# Autodesk Inventor assembly: Channel
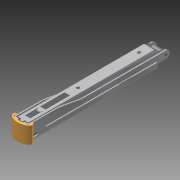
[picture p0: Inventor's stored thumbnail of the model, 180x180]
Saved by Autodesk Inventor 2011 (Build 150239000, 239)
## iProperties
Shininess: 64.0
Length Units: 11272
Angle Units: 11279
Time Units: 11290
Mass Units: 11286
Length Display Precision: 3
Angle Display Precision: 2
Compacted: True
Part Number: Channel
Document SubType Name: Assembly
Created: 2002-09-26
Designer: Autodesk, Inc.
Project: Inventor Samples
Mass: 81.6929 g
Surface Area: 254.71 cm^2
Volume: 11.1757 cm^3
Density: 7.30984 g/cm^3
Density: 0.0
Volumn: 0.0
Area: 0.0
PropertySet Name: Model Information
Control State: 0
Master: False
Checked Out: False
Author: Autodesk, Inc.
Revision Number: A
## Documents named in this file (7)
- C:\Users\Public\Documents\Autodesk\Inventor 2011\Samples\Models\Assemblies\Stapler\Components\Channel.iam
- C:\Users\Public\Documents\Autodesk\Inventor 2011\Samples\Models\Assemblies\Stapler\Components\Channel - Base.ipt
- C:\Users\Public\Documents\Autodesk\Inventor 2011\Samples\Models\Assemblies\Stapler\Components\Channel - Pusher.ipt
- C:\Users\Public\Documents\Autodesk\Inventor 2011\Samples\Models\Assemblies\Stapler\Components\Channel - Cover.ipt
- C:\Users\Public\Documents\Autodesk\Inventor 2011\Samples\Models\Assemblies\Stapler\Components\Channel - Hinge Pin.ipt
- C:\Users\Public\Documents\Autodesk\Inventor 2011\Samples\Models\Assemblies\Stapler\Components\Staples.ipt
- C:\Users\Public\Documents\Autodesk\Inventor 2011\Samples\Models\Assemblies\Stapler\Components\Channel - Bumper.ipt
## Components (6 placed, 6 different names)
1. Channel - Base:1 — Mate:1, Flush:1, Flush:2, Flush:3, Tangent:1, Flush:5, Mate:3, Mate:4, Flush:7, Mate:6, Mate:7
2. Channel - Pusher:1 — Mate:1, Flush:1, Mate:5
3. Channel - Cover:1 — Flush:2, Flush:3, Tangent:1, Mate:2
4. Channel - Hinge Pin:1 — Flush:4, Mate:2, Flush:5
5. Staples:1 — Mate:3, Flush:6, Mate:4, Mate:5
6. Channel - Bumper:1 — Flush:7, Mate:6, Mate:7
## Relationships (15: Mate 7, Flush 7, Tangent 1)
- Mate:1: Channel - Base:1 ↔ Channel - Pusher:1
- Flush:1: Channel - Base:1 ↔ Channel - Pusher:1
- Flush:2: Channel - Base:1 ↔ Channel - Cover:1
- Flush:3: Channel - Base:1 ↔ Channel - Cover:1
- Tangent:1: Channel - Base:1 ↔ Channel - Cover:1
- Flush:4: Channel - Hinge Pin:1
- Mate:2: Channel - Cover:1 ↔ Channel - Hinge Pin:1
- Flush:5: Channel - Base:1 ↔ Channel - Hinge Pin:1
- Mate:3: Channel - Base:1 ↔ Staples:1
- Flush:6: Staples:1
- Mate:4: Channel - Base:1 ↔ Staples:1
- Mate:5: Channel - Pusher:1 ↔ Staples:1
- Flush:7: Channel - Base:1 ↔ Channel - Bumper:1
- Mate:6: Channel - Base:1 ↔ Channel - Bumper:1
- Mate:7: Channel - Base:1 ↔ Channel - Bumper:1
